# Autodesk Inventor assembly: DeliveryArmWithServo
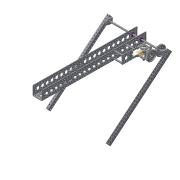
[picture p0: Inventor's stored thumbnail of the model, 180x180]
Saved by Autodesk Inventor 2018 (Build 220112000, 112)
## iProperties
Created: 2018-10-26
Part Number: DeliveryArmWithServo
Document SubType Name: Assembly
Designer: ball
Author: ball
## Documents named in this file (8)
- C:\FTC\FTC8863CAD\2018Robot\DeliveryArmWithServo.iam
- C:\FTC\FTC8863CAD\Actobotics\585 parts\585460.ipt
- C:\FTC\FTC8863CAD\Actobotics\535 parts\535198.ipt
- C:\FTC\FTC8863CAD\2018Robot\ServoBlockLargeServoPlateWithStandoffs.iam
- C:\FTC\FTC8863CAD\Actobotics\615 parts\615190.ipt
- C:\FTC\FTC8863CAD\Actobotics\545 parts\545619 assembly.ipt
- C:\FTC\FTC8863CAD\Actobotics\634 parts\634090.ipt
- C:\FTC\FTC8863CAD\2018Robot\DeliveryDropArm.iam
## Components (10 placed, 7 different names)
1. 585460:1 — Mate:1, Mate:2, Mate:3, Mate:4, Mate:5, Mate:6, Mate:7, Mate:18
2. 535198:1 — Mate:1, Mate:2, Mate:15
3. 535198:2 — Mate:3, Mate:4
4. ServoBlockLargeServoPlateWithStandoffs:1 [sub-assembly] — Mate:5, Mate:6, Mate:7, Mate:8, Mate:9, Mate:10
5. 615190:2 — Mate:8, Mate:9, Mate:10, Flush:1
6. 615190:3 — Mate:12, Mate:13, Mate:14, Flush:1
7. 545619 assembly:3 — Mate:12, Mate:13, Mate:14, Mate:16
8. 634090:1 — Mate:15, Mate:16, Mate:17, Flush:2, Mate:19, Flush:3
9. DeliveryDropArm:2 [sub-assembly] — Mate:17, Flush:2, Mate:18, Angle:1
10. DeliveryDropArm:4 [sub-assembly] — Mate:19, Flush:3, Angle:1
## Relationships (22: Mate 18, Flush 3, Angle 1)
- Mate:1: 585460:1 ↔ 535198:1
- Mate:2: 585460:1 ↔ 535198:1
- Mate:3: 585460:1 ↔ 535198:2
- Mate:4: 585460:1 ↔ 535198:2
- Mate:5: 585460:1 ↔ ServoBlockLargeServoPlateWithStandoffs:1
- Mate:6: 585460:1 ↔ ServoBlockLargeServoPlateWithStandoffs:1
- Mate:7: 585460:1 ↔ ServoBlockLargeServoPlateWithStandoffs:1
- Mate:8: ServoBlockLargeServoPlateWithStandoffs:1 ↔ 615190:2
- Mate:9: ServoBlockLargeServoPlateWithStandoffs:1 ↔ 615190:2
- Mate:10: ServoBlockLargeServoPlateWithStandoffs:1 ↔ 615190:2
- Mate:12: 615190:3 ↔ 545619 assembly:3
- Mate:13: 615190:3 ↔ 545619 assembly:3
- Mate:14: 615190:3 ↔ 545619 assembly:3
- Mate:15: 535198:1 ↔ 634090:1
- Mate:16: 545619 assembly:3 ↔ 634090:1
- Flush:1: 615190:2 ↔ 615190:3
- Mate:17: 634090:1 ↔ DeliveryDropArm:2
- Flush:2: 634090:1 ↔ DeliveryDropArm:2
- Mate:18 (88.265 mm): 585460:1 ↔ DeliveryDropArm:2
- Mate:19: 634090:1 ↔ DeliveryDropArm:4
- Flush:3: 634090:1 ↔ DeliveryDropArm:4
- Angle:1 (0 deg): DeliveryDropArm:2 ↔ DeliveryDropArm:4
